# Autodesk Inventor assembly: Z Extrusion Left
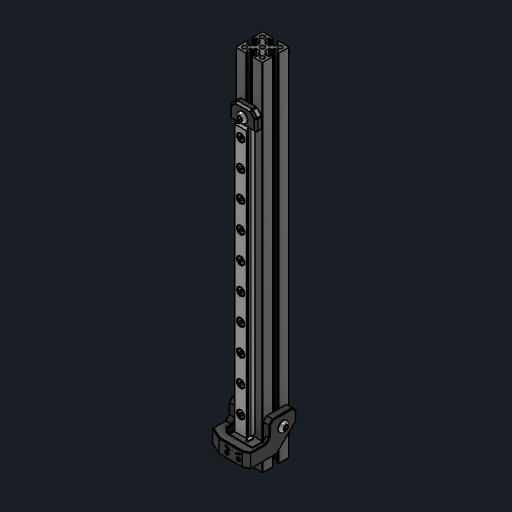
[picture p0: Inventor's stored thumbnail of the model, 512x512]
Saved by Autodesk Inventor 2026 (Build 300175050, 175E)
## iProperties
Created: 2025-05-11
Part Number: Z Extrusion Left
Document SubType Name: Assembly
Designer: Joshua Eah
Author: Joshua Eah
## Documents named in this file (8)
- C:\Users\Joshua Eah\Documents\GitHub\Voron-0\CAD\Master Assembly\Z Axis\Z Extrusion Left.iam
- C:\Users\Joshua Eah\Documents\GitHub\Voron-0\CAD\Master Assembly\Frame\Parts\1515_200mm - C.ipt
- C:\Users\Joshua Eah\Documents\GitHub\Voron-0\CAD\Master Assembly\Hardware\M3x6 BHCS.ipt
- C:\Users\Joshua Eah\Documents\GitHub\Voron-0\CAD\Master Assembly\Hardware\M3 Hexnut.ipt
- C:\Users\Joshua Eah\Documents\GitHub\Voron-0\CAD\Master Assembly\Linear Rail\MGN7 Rail 150mm.iam
- MGN7 150mm Rail.iam
- C:\Users\Joshua Eah\Documents\GitHub\Voron-0\CAD\Master Assembly\Z Axis\Z Endstop Assembly.iam
- C:\Users\Joshua Eah\Documents\GitHub\Voron-0\CAD\Master Assembly\Frame\Subassemblies\Rail Stop.iam
## Components (8 placed, 6 different names)
1. 1515_200mm - C:3
2. MGN7 Rail 150mm:1 [sub-assembly]
3. Rail Stop:1 [sub-assembly]
4. Z Endstop Assembly:1 [sub-assembly]
5. M3x6 BHCS:1
6. M3x6 BHCS:2
7. M3 Hexnut:6
8. M3 Hexnut:7
## Relationships (15: Mate 11, Insert 2, Flush 2)
- [Mate]: 1515_200mm - C:3 ↔ M3x6 BHCS:1
- [Mate]: 1515_200mm - C:3 ↔ M3x6 BHCS:1
- [Mate]: 1515_200mm - C:3 ↔ M3x6 BHCS:2
- [Mate]: 1515_200mm - C:3 ↔ M3x6 BHCS:2
- [Insert]: M3x6 BHCS:1 ↔ M3 Hexnut:7
- [Insert]: M3x6 BHCS:2 ↔ M3 Hexnut:6
- [Mate]: 1515_200mm - C:3 ↔ MGN7 Rail 150mm:1
- [Flush] (33 mm): 1515_200mm - C:3 ↔ MGN7 Rail 150mm:1
- [Mate] (0.1 mm): 1515_200mm - C:3 ↔ MGN7 Rail 150mm:1
- [Mate]: MGN7 Rail 150mm:1 ↔ Rail Stop:1
- [Mate]: 1515_200mm - C:3 ↔ Rail Stop:1
- [Flush]: 1515_200mm - C:3 ↔ Rail Stop:1
- [Mate]: MGN7 Rail 150mm:1 ↔ Z Endstop Assembly:1
- [Mate]: 1515_200mm - C:3 ↔ Z Endstop Assembly:1
- [Mate]: 1515_200mm - C:3 ↔ Z Endstop Assembly:1
## Named parameters: d0_d2 = 0 mm, d1_d3 = 0 mm, d6_d10 = 0 mm
